# Autodesk Inventor assembly: PMax4
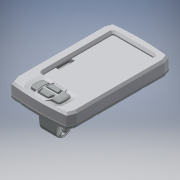
[picture p0: Inventor's stored thumbnail of the model, 180x180]
Saved by Autodesk Inventor 2018 (Build 220112000, 112)
## iProperties
Created: 2019-05-29
Part Number: PMax4
Document SubType Name: Assembly
Designer: Ash
Author: Ash
## Documents named in this file (7)
- C:\Autodesk\Skills 2019 Nationals\Competition\PMDay2\PMax4.iam
- C:\Autodesk\Skills 2019 Nationals\Competition\PMDay2\#2-KEYPAD.ipt
- C:\Autodesk\Skills 2019 Nationals\Competition\PMDay2\#5-BACK_COVER(PMAX4).ipt
- C:\Autodesk\Skills 2019 Nationals\Competition\PMDay2\#6-SCREW.ipt
- C:\Autodesk\Skills 2019 Nationals\Competition\PMDay1\Display_Plate.ipt
- C:\Autodesk\Skills 2019 Nationals\Competition\PMDay1\Front_Cover.ipt
- C:\Autodesk\Skills 2019 Nationals\Competition\PMDay2\#4-GASKET(PMAX4) copy.ipt
## Components (13 placed, 6 different names)
1. #2-KEYPAD:1 — Mate:6, Mate:7, Mate:8, Mate:9, Mate:11
2. #4-GASKET(PMAX4) copy:1 — Mate:1, Mate:2, Mate:3
3. #5-BACK_COVER(PMAX4):1 — Mate:1, Mate:2, Mate:3, Mate:4, Mate:5, Mate:12, Mate:13, Mate:14, Mate:15, Mate:16, Mate:17, Mate:18, Mate:19, Mate:20, Mate:21, Mate:22, Mate:23, Mate:24, Mate:25, Mate:26, Mate:27, Mate:28
4. #6-SCREW:1 — Mate:13, Mate:22
5. #6-SCREW:2 — Mate:20, Mate:21
6. #6-SCREW:3 — Mate:19, Mate:28
7. #6-SCREW:4 — Mate:18, Mate:27
8. #6-SCREW:5 — Mate:14, Mate:23
9. #6-SCREW:6 — Mate:15, Mate:24
10. #6-SCREW:7 — Mate:16, Mate:25
11. #6-SCREW:8 — Mate:17, Mate:26
12. Display_Plate:1 — Mate:7, Mate:10, Mate:11
13. Front_Cover:1 — Mate:4, Mate:5, Mate:6, Mate:8, Mate:9, Mate:10, Mate:12
## Relationships (28: Mate 28)
- Mate:1: #4-GASKET(PMAX4) copy:1 ↔ #5-BACK_COVER(PMAX4):1
- Mate:2: #4-GASKET(PMAX4) copy:1 ↔ #5-BACK_COVER(PMAX4):1
- Mate:3: #4-GASKET(PMAX4) copy:1 ↔ #5-BACK_COVER(PMAX4):1
- Mate:4: #5-BACK_COVER(PMAX4):1 ↔ Front_Cover:1
- Mate:5: #5-BACK_COVER(PMAX4):1 ↔ Front_Cover:1
- Mate:6 (6.35 mm): #2-KEYPAD:1 ↔ Front_Cover:1
- Mate:7: #2-KEYPAD:1 ↔ Display_Plate:1
- Mate:8: #2-KEYPAD:1 ↔ Front_Cover:1
- Mate:9 (46.7868 mm): #2-KEYPAD:1 ↔ Front_Cover:1
- Mate:10: Display_Plate:1 ↔ Front_Cover:1
- Mate:11: #2-KEYPAD:1 ↔ Display_Plate:1
- Mate:12: #5-BACK_COVER(PMAX4):1 ↔ Front_Cover:1
- Mate:13: #5-BACK_COVER(PMAX4):1 ↔ #6-SCREW:1
- Mate:14: #5-BACK_COVER(PMAX4):1 ↔ #6-SCREW:5
- Mate:15: #5-BACK_COVER(PMAX4):1 ↔ #6-SCREW:6
- Mate:16: #5-BACK_COVER(PMAX4):1 ↔ #6-SCREW:7
- Mate:17: #5-BACK_COVER(PMAX4):1 ↔ #6-SCREW:8
- Mate:18: #5-BACK_COVER(PMAX4):1 ↔ #6-SCREW:4
- Mate:19: #5-BACK_COVER(PMAX4):1 ↔ #6-SCREW:3
- Mate:20: #5-BACK_COVER(PMAX4):1 ↔ #6-SCREW:2
- Mate:21: #5-BACK_COVER(PMAX4):1 ↔ #6-SCREW:2
- Mate:22: #5-BACK_COVER(PMAX4):1 ↔ #6-SCREW:1
- Mate:23: #5-BACK_COVER(PMAX4):1 ↔ #6-SCREW:5
- Mate:24: #5-BACK_COVER(PMAX4):1 ↔ #6-SCREW:6
- Mate:25: #5-BACK_COVER(PMAX4):1 ↔ #6-SCREW:7
- Mate:26: #5-BACK_COVER(PMAX4):1 ↔ #6-SCREW:8
- Mate:27: #5-BACK_COVER(PMAX4):1 ↔ #6-SCREW:4
- Mate:28: #5-BACK_COVER(PMAX4):1 ↔ #6-SCREW:3
